# Autodesk Inventor assembly: MG-Akku 6S1P
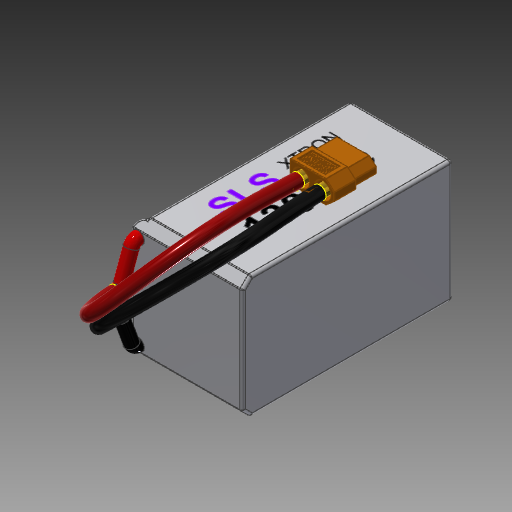
[picture p0: Inventor's stored thumbnail of the model, 512x512]
Saved by Autodesk Inventor 2019.4 (Build 234330000, 330)
## iProperties
Part Number: MG-Akku 6S1P
Material: Generisch
Document SubType Name: Assembly
Designer: rYan
Mass: 251.621 g
Surface Area: 167.344 cm^2
Volume: 116.033 cm^3
Density: 2.16853 g/cm^3
Author: rYan
## Documents named in this file (4)
- D:\TIGERsGIT\Hardware\mechanik\2020\Inventor\Purchased Parts\MG-Akku 6S1P.iam
- D:\TIGERsGIT\Hardware\mechanik\2020\Inventor\Purchased Parts\Akku 6S1P SLS Goblin Fireball.ipt
- D:\TIGERsGIT\Hardware\mechanik\2020\Inventor\Purchased Parts\XT60 Buchse.ipt
- D:\TIGERsGIT\Hardware\mechanik\2020\Inventor\Purchased Parts\MG-Akku 6S1P\AIP\Kabel und Kabelbaum\MG-Akku 6S1P.Kabelbaum.iam
## Components (3 placed, 3 different names)
1. Akku 6S1P SLS Goblin Fireball:1 — Passend:1, Passend:2
2. XT60 Buchse:1 — Passend:1, Passend:2
3. MG-Akku 6S1P.Kabelbaum [sub-assembly]
## Relationships (2: Mate 2)
- Passend:1 [Mate] (5 mm): Akku 6S1P SLS Goblin Fireball:1 ↔ XT60 Buchse:1
- Passend:2 [Mate] (2 mm): Akku 6S1P SLS Goblin Fireball:1 ↔ XT60 Buchse:1
